# Autodesk Inventor assembly: POM_T5_05
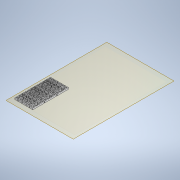
[picture p0: Inventor's stored thumbnail of the model, 180x180]
Saved by Autodesk Inventor 2022 (Build 260153000, 153)
## iProperties
Created: 2022-09-28
Part Number: POM_T5_05
Document SubType Name: Assembly
Designer: Masato
Author: Masato
## Documents named in this file (3)
- C:\Users\ヨコオリク\Documents\CITBrains\SUSTAINA-OP\Cam\POM_T5\OriginalMind_SR420\POM_T5_05.iam
- C:\Users\ヨコオリク\Documents\CITBrains\SUSTAINA-OP\Cam\DisposableBoard.ipt
- C:\Users\ヨコオリク\Documents\CITBrains\SUSTAINA-OP\OptionParts\DrillingJigs\UpperArm_diagonal_Jig.ipt
## Components (16 placed, 2 different names)
1. DisposableBoard:1 — フラッシュ:1, フラッシュ:2, フラッシュ:3, フラッシュ:4, フラッシュ:5, フラッシュ:6
2. UpperArm_diagonal_Jig:1 — メイト:1, フラッシュ:5, フラッシュ:6
3. UpperArm_diagonal_Jig:2
4. UpperArm_diagonal_Jig:3
5. UpperArm_diagonal_Jig:4
6. UpperArm_diagonal_Jig:5
7. UpperArm_diagonal_Jig:6
8. UpperArm_diagonal_Jig:7
9. UpperArm_diagonal_Jig:8
10. UpperArm_diagonal_Jig:9
11. UpperArm_diagonal_Jig:10
12. UpperArm_diagonal_Jig:11
13. UpperArm_diagonal_Jig:12
14. UpperArm_diagonal_Jig:13
15. UpperArm_diagonal_Jig:14
16. UpperArm_diagonal_Jig:15
## Component patterns: (15 elements, first: UpperArm_diagonal_Jig:1)
## Relationships (7: Flush 6, Mate 1)
- フラッシュ:1 [Flush]: DisposableBoard:1
- フラッシュ:2 [Flush]: DisposableBoard:1
- フラッシュ:3 [Flush]: DisposableBoard:1
- フラッシュ:4 [Flush]: DisposableBoard:1
- メイト:1 [Mate]: UpperArm_diagonal_Jig:1
- フラッシュ:5 [Flush] (2 mm): DisposableBoard:1 ↔ UpperArm_diagonal_Jig:1
- フラッシュ:6 [Flush] (2 mm): DisposableBoard:1 ↔ UpperArm_diagonal_Jig:1
